# Autodesk Inventor assembly: tail_p3
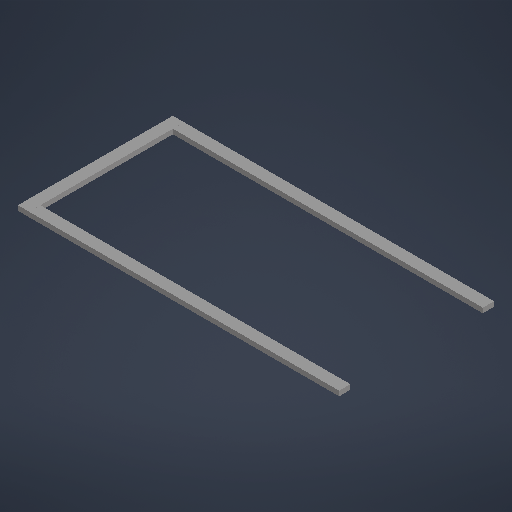
[picture p0: Inventor's stored thumbnail of the model, 512x512]
Saved by Autodesk Inventor 2027.1 (Build 311270010, 270A)
## iProperties
Created: 2026-09-01
Part Number: tail_p3
Document SubType Name: Assembly
Designer: jorda
Author: jorda
## Documents named in this file (3)
- C:\Users\jorda\OneDrive\Documents\GitHub\USC-ASME-TigerBurn-2026\CAD\Tail\tail_p3.iam
- C:\Users\jorda\OneDrive\Documents\GitHub\USC-ASME-TigerBurn-2026\CAD\Tail\2x4x48.ipt
- C:\Users\jorda\OneDrive\Documents\GitHub\USC-ASME-TigerBurn-2026\CAD\Tail\2x4x96.ipt
## Components (3 placed, 2 different names)
1. 2x4x48:1 — Mate:1, Flush:1, Flush:2, Mate:2, Flush:3, Flush:4
2. 2x4x96:1 — Mate:1, Flush:1, Flush:2
3. 2x4x96:2 — Mate:2, Flush:3, Flush:4
## Relationships (6: Flush 4, Mate 2)
- Mate:1: 2x4x48:1 ↔ 2x4x96:1
- Flush:1: 2x4x48:1 ↔ 2x4x96:1
- Flush:2: 2x4x48:1 ↔ 2x4x96:1
- Mate:2: 2x4x48:1 ↔ 2x4x96:2
- Flush:3: 2x4x48:1 ↔ 2x4x96:2
- Flush:4: 2x4x48:1 ↔ 2x4x96:2
